# Autodesk Inventor assembly: FE-00001
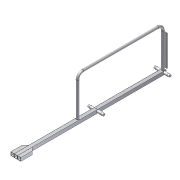
[picture p0: Inventor's stored thumbnail of the model, 180x180]
Saved by Autodesk Inventor 2012 (Build 160160000, 160)
## iProperties
Created: 2008-05-14
Part Number: FE-00001
Document SubType Name: Assembly
Designer: narosenberg
Mass: 2481.09 g
Surface Area: 12809.7 cm^2
Volume: 2481.09 cm^3
Density: 1 g/cm^3
Description: Driver's Station Support Assy
Author: narosenberg
## Documents named in this file (6)
- C:\Data Folder\FRC 2012 Field\Components\FE-00001.iam
- C:\Data Folder\FRC 2012 Field\Components\FE-00001-01.ipt
- C:\Data Folder\FRC 2012 Field\Components\FE-00001-02.ipt
- C:\Data Folder\FRC 2012 Field\Components\FE-00001-03.ipt
- C:\Data Folder\FRC 2012 Field\Components\FE-00001-04.ipt
- C:\Data Folder\FRC 2012 Field\Components\FE-00001-05.ipt
## Components (7 placed, 5 different names)
1. FE-00001-05:1 — Insert:1, Insert:2, Mate:1, Angle:1, Mate:3, Angle:2, Angle:3, Mate:4, Mate:5, Flush:1, Mate:6, Mate:7, Mate:8, Mate:9
2. FE-00001-04:1 — Insert:1
3. FE-00001-04:2 — Insert:2
4. FE-00001-03:1 — Mate:1, Angle:1, Mate:2, Mate:3, Tangent:1
5. FE-00001-02:1 — Angle:2, Angle:3, Mate:4, Tangent:1, Mate:5, Flush:1
6. FE-00001-01:2 — Mate:8, Mate:9
7. FE-00001-01:1 — Mate:6, Mate:7
## Relationships (16: Mate 9, Angle 3, Insert 2, Tangent 1, Flush 1)
- Insert:1 (-82.55 mm): FE-00001-05:1 ↔ FE-00001-04:1
- Insert:2 (-76.2 mm): FE-00001-05:1 ↔ FE-00001-04:2
- Mate:1: FE-00001-05:1 ↔ FE-00001-03:1
- Angle:1 (0 deg): FE-00001-05:1 ↔ FE-00001-03:1
- Mate:2: FE-00001-03:1
- Mate:3: FE-00001-05:1 ↔ FE-00001-03:1
- Angle:2 (0 deg): FE-00001-05:1 ↔ FE-00001-02:1
- Angle:3 (0 deg): FE-00001-05:1 ↔ FE-00001-02:1
- Mate:4: FE-00001-05:1 ↔ FE-00001-02:1
- Tangent:1: FE-00001-03:1 ↔ FE-00001-02:1
- Mate:5 (25.4 mm): FE-00001-05:1 ↔ FE-00001-02:1
- Flush:1: FE-00001-05:1 ↔ FE-00001-02:1
- Mate:6: FE-00001-05:1 ↔ FE-00001-01:1
- Mate:7: FE-00001-05:1 ↔ FE-00001-01:1
- Mate:8: FE-00001-05:1 ↔ FE-00001-01:2
- Mate:9: FE-00001-05:1 ↔ FE-00001-01:2
